# Autodesk Inventor assembly: new subsystem 1 assembly
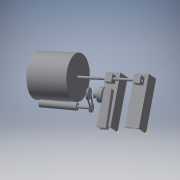
[picture p0: Inventor's stored thumbnail of the model, 180x180]
Saved by Autodesk Inventor 2019 (Build 230136000, 136)
## iProperties
Created: 2020-03-05
Part Number: new subsystem 1 assembly
Document SubType Name: Assembly
Designer: User
Author: User
## Documents named in this file (5)
- C:\Users\User\Desktop\assembly\Assembly  ss1.iam
- C:\Users\User\Desktop\Subsystem 1\Kettle.ipt
- C:\Users\User\Desktop\Subsystem 1\rod 1.ipt
- C:\Users\User\Desktop\Subsystem 1\stand 1.ipt
- C:\Users\User\Desktop\Subsystem 1\Assembly2.iam
## Components (5 placed, 4 different names)
1. Kettle:1 — Rotational:1
2. rod 1:1 — Rotational:1, Rigid:1, Rotational:2
3. stand 1:1 — Rigid:1
4. stand 1:2 — Rotational:2
5. Assembly2:1 [sub-assembly]
## Relationships (3: RevoluteJoint 2, WeldJoint 1)
- Rotational:1 [RevoluteJoint]: Kettle:1 ↔ rod 1:1
- Rigid:1 [WeldJoint]: rod 1:1 ↔ stand 1:1
- Rotational:2 [RevoluteJoint]: rod 1:1 ↔ stand 1:2
